# Autodesk Inventor assembly: calosc
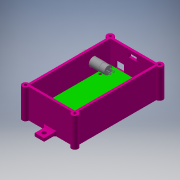
[picture p0: Inventor's stored thumbnail of the model, 180x180]
Saved by Autodesk Inventor 2019 (Build 230136000, 136)
## iProperties
Created: 2019-09-16
Part Number: calosc
Material: Ogólny
Document SubType Name: Assembly
Designer: mikol
Author: mikol
## Documents named in this file (5)
- C:\Users\mikol\Desktop\Projekty\Pomiar_poziomu_wody\baza\projekt_obudowy\calosc.iam
- C:\Users\mikol\Desktop\Projekty\Pomiar_poziomu_wody\baza\projekt_obudowy\Podstawa.ipt
- C:\Users\mikol\Desktop\Projekty\Pomiar_poziomu_wody\baza\projekt_obudowy\PCB.ipt
- C:\Users\mikol\Desktop\Projekty\Pomiar_poziomu_wody\baza\projekt_obudowy\gora.ipt
- C:\Users\mikol\Desktop\Projekty\Pomiar_poziomu_wody\baza\projekt_obudowy\przycisk.ipt
## Components (4 placed, 4 different names)
1. Podstawa:1 — Rigid:1, Rigid:2, Rigid:3
2. PCB:1 — Rigid:1
3. gora:1 — Rigid:2
4. przycisk:1 — Rigid:3
## Relationships (3: WeldJoint 3)
- Rigid:1 [WeldJoint]: Podstawa:1 ↔ PCB:1
- Rigid:2 [WeldJoint] (-1 mm): Podstawa:1 ↔ gora:1
- Rigid:3 [WeldJoint]: Podstawa:1 ↔ przycisk:1
